# Autodesk Inventor assembly: Rod Support for Constant Force Springs
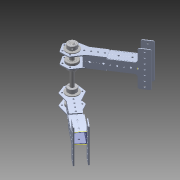
[picture p0: Inventor's stored thumbnail of the model, 180x180]
Saved by Autodesk Inventor 2014 (Build 180170000, 170)
## iProperties
Created: 2014-01-07
Part Number: Rod Support for Constant Force Springs
Document SubType Name: Assembly
Designer: Michael
Author: Michael
## Documents named in this file (7)
- C:\Users\Michael\Documents\GitHub\2014buildCAD\Funnel Catcher\Rod Support for Constant Force Springs.iam
- C:\Users\Michael\Documents\GitHub\2014buildCAD\Funnel Catcher\Vex Pro End Bearing Mount.ipt
- C:\Users\Michael\Documents\GitHub\2014buildCAD\Funnel Catcher\Vex Pro 1x1 rectangular tubing 4 in length.ipt
- C:\Users\Michael\Documents\GitHub\2014buildCAD\Funnel Catcher\3-8 ID 1.125 OD Bearing (6384K348).ipt
- C:\Users\Michael\Documents\GitHub\2014buildCAD\Funnel Catcher\6 in 3-8 diameter Shaft (6061K120).ipt
- C:\Users\Michael\Documents\GitHub\2014buildCAD\Funnel Catcher\3-8 in ID shaft collar (6435K130).ipt
- C:\Users\Michael\Documents\GitHub\2014buildCAD\Funnel Catcher\Vex Pro T Gusset.ipt
## Components (19 placed, 6 different names)
1. Vex Pro End Bearing Mount:1
2. Vex Pro 1x1 rectangular tubing 4 in length:1 — Insert:21, Insert:22, Insert:23, Insert:24, Insert:25
3. Vex Pro End Bearing Mount:2 — Insert:25
4. 3-8 ID 1.125 OD Bearing (6384K348):1 — Insert:8
5. 3-8 ID 1.125 OD Bearing (6384K348):2 — Insert:7
6. 6 in 3-8 diameter Shaft (6061K120):1 — Insert:6, Insert:14
7. 3-8 in ID shaft collar (6435K130):1 — Insert:6, Insert:7
8. 3-8 in ID shaft collar (6435K130):2 — Insert:14, Insert:15
9. 3-8 in ID shaft collar (6435K130):3 — Insert:16
10. 3-8 in ID shaft collar (6435K130):4 — Insert:8
11. Vex Pro End Bearing Mount:3
12. Vex Pro 1x1 rectangular tubing 4 in length:2 — Insert:17, Insert:18, Insert:19, Insert:20, Insert:26
13. Vex Pro End Bearing Mount:4 — Insert:26
14. 3-8 ID 1.125 OD Bearing (6384K348):3 — Insert:15
15. 3-8 ID 1.125 OD Bearing (6384K348):4 — Insert:16
16. Vex Pro T Gusset:1 — Insert:17, Insert:18
17. Vex Pro T Gusset:2 — Insert:23, Insert:24
18. Vex Pro T Gusset:3 — Insert:21, Insert:22
19. Vex Pro T Gusset:4 — Insert:19, Insert:20
## Relationships (26: Insert 26)
- [Insert]: Vex Pro End Bearing Mount:2 ↔ 3-8 ID 1.125 OD Bearing (6384K348):2
- [Insert]: Vex Pro End Bearing Mount:1 ↔ 3-8 ID 1.125 OD Bearing (6384K348):1
- [Insert]: Vex Pro End Bearing Mount:1 ↔ Vex Pro 1x1 rectangular tubing 4 in length:1
- [Insert]: Vex Pro 1x1 rectangular tubing 4 in length:1 ↔ Vex Pro End Bearing Mount:2
- [Insert]: Vex Pro End Bearing Mount:1 ↔ Vex Pro 1x1 rectangular tubing 4 in length:1
- Insert:6: 6 in 3-8 diameter Shaft (6061K120):1 ↔ 3-8 in ID shaft collar (6435K130):1
- Insert:7: 3-8 ID 1.125 OD Bearing (6384K348):2 ↔ 3-8 in ID shaft collar (6435K130):1
- Insert:8: 3-8 ID 1.125 OD Bearing (6384K348):1 ↔ 3-8 in ID shaft collar (6435K130):4
- [Insert]: Vex Pro End Bearing Mount:4 ↔ 3-8 ID 1.125 OD Bearing (6384K348):4
- [Insert]: Vex Pro End Bearing Mount:3 ↔ 3-8 ID 1.125 OD Bearing (6384K348):3
- [Insert]: Vex Pro End Bearing Mount:3 ↔ Vex Pro 1x1 rectangular tubing 4 in length:2
- [Insert]: Vex Pro 1x1 rectangular tubing 4 in length:2 ↔ Vex Pro End Bearing Mount:4
- [Insert]: Vex Pro End Bearing Mount:3 ↔ Vex Pro 1x1 rectangular tubing 4 in length:2
- Insert:14: 6 in 3-8 diameter Shaft (6061K120):1 ↔ 3-8 in ID shaft collar (6435K130):2
- Insert:15: 3-8 in ID shaft collar (6435K130):2 ↔ 3-8 ID 1.125 OD Bearing (6384K348):3
- Insert:16: 3-8 in ID shaft collar (6435K130):3 ↔ 3-8 ID 1.125 OD Bearing (6384K348):4
- Insert:17: Vex Pro 1x1 rectangular tubing 4 in length:2 ↔ Vex Pro T Gusset:1
- Insert:18: Vex Pro 1x1 rectangular tubing 4 in length:2 ↔ Vex Pro T Gusset:1
- Insert:19: Vex Pro 1x1 rectangular tubing 4 in length:2 ↔ Vex Pro T Gusset:4
- Insert:20: Vex Pro 1x1 rectangular tubing 4 in length:2 ↔ Vex Pro T Gusset:4
- Insert:21: Vex Pro 1x1 rectangular tubing 4 in length:1 ↔ Vex Pro T Gusset:3
- Insert:22: Vex Pro 1x1 rectangular tubing 4 in length:1 ↔ Vex Pro T Gusset:3
- Insert:23: Vex Pro 1x1 rectangular tubing 4 in length:1 ↔ Vex Pro T Gusset:2
- Insert:24: Vex Pro 1x1 rectangular tubing 4 in length:1 ↔ Vex Pro T Gusset:2
- Insert:25: Vex Pro 1x1 rectangular tubing 4 in length:1 ↔ Vex Pro End Bearing Mount:2
- Insert:26: Vex Pro 1x1 rectangular tubing 4 in length:2 ↔ Vex Pro End Bearing Mount:4
## Named parameters: d3_d4 = 0 mm, d9_d30 = 0 mm, d10_d31 = 0 mm, d11_d32 = 0 mm, d12_d3_d4 = 0 mm, d13_d5 = 0 mm
